# Autodesk Inventor assembly: robot
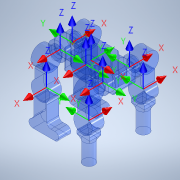
[picture p0: Inventor's stored thumbnail of the model, 180x180]
Saved by Autodesk Inventor 2020.2 (Build 242310000, 310)
## iProperties
Created: 2021-01-29
Part Number: robot
Document SubType Name: Assembly
Designer: DELL
Author: DELL
## Documents named in this file (6)
- D:\repo\FlexipodFast\mesh\v8.0\robot.iam
- D:\repo\FlexipodFast\mesh\v8.0\body.ipt
- D:\repo\FlexipodFast\mesh\v8.0\hip.ipt
- D:\repo\FlexipodFast\mesh\v8.0\thigh.ipt
- D:\repo\FlexipodFast\mesh\v8.0\shank_2.ipt
- D:\repo\FlexipodFast\mesh\v8.0\shank_front.ipt
## Components (13 placed, 5 different names)
1. body:1 — Flush:1, Flush:2, Flush:3, Mate:1, Mate:2, Mate:3, Mate:4, Angle:4, Angle:6, Angle:15, Angle:16, Angle:17, Angle:18, Mate:45, Mate:46, Mate:48, Mate:49, Angle:19, Angle:20, Angle:21, Angle:23, Angle:24, Angle:25, Angle:26, Angle:27, Angle:28, Angle:29, Angle:30, Angle:31
2. hip:1 — Mate:3, Mate:4, Angle:30, Flush:45, Mate:54
3. hip:2 — Mate:1, Mate:2, Angle:22, Angle:29, Mate:52, Mate:53
4. thigh:1 — Angle:17, Mate:44, Flush:43, Mate:52, Mate:53
5. thigh:2 — Angle:6, Mate:43, Flush:42, Angle:19, Angle:20, Flush:45, Mate:54
6. thigh:3 — Angle:16, Mate:42, Flush:41, Angle:23, Angle:24, Mate:55, Mate:56
7. thigh:4 — Angle:4, Angle:15, Angle:18, Mate:41, Flush:40, Angle:25, Angle:26, Mate:57, Flush:46
8. shank_2:3 — Mate:41, Flush:40, Angle:27
9. shank_2:4 — Mate:42, Flush:41, Angle:28
10. shank_front:1 — Mate:43, Flush:42, Angle:21
11. shank_front:2 — Mate:44, Flush:43, Angle:22
12. hip:3 — Mate:45, Mate:46, Mate:55, Angle:31, Mate:56
13. hip:4 — Mate:48, Mate:49, Mate:57, Flush:46
## Relationships (46: Angle 19, Mate 18, Flush 9)
- Flush:1: body:1
- Flush:2: body:1
- Flush:3: body:1
- Mate:1: body:1 ↔ hip:2
- Mate:2: body:1 ↔ hip:2
- Mate:3: body:1 ↔ hip:1
- Mate:4: body:1 ↔ hip:1
- Angle:4 (0 deg): body:1 ↔ thigh:4
- Angle:6 (0 deg): body:1 ↔ thigh:2
- Angle:15 (0 deg): body:1 ↔ thigh:4
- Angle:16 (0 deg): body:1 ↔ thigh:3
- Angle:17 (0 deg): body:1 ↔ thigh:1
- Angle:18 (0 deg): body:1 ↔ thigh:4
- Mate:41: thigh:4 ↔ shank_2:3
- Flush:40: thigh:4 ↔ shank_2:3
- Mate:42: thigh:3 ↔ shank_2:4
- Flush:41: thigh:3 ↔ shank_2:4
- Mate:43: thigh:2 ↔ shank_front:1
- Mate:44: thigh:1 ↔ shank_front:2
- Flush:42: thigh:2 ↔ shank_front:1
- Flush:43: thigh:1 ↔ shank_front:2
- Mate:45: body:1 ↔ hip:3
- Mate:46: body:1 ↔ hip:3
- Mate:48: body:1 ↔ hip:4
- Mate:49: body:1 ↔ hip:4
- Angle:19 (0 deg): body:1 ↔ thigh:2
- Angle:20 (0 deg): body:1 ↔ thigh:2
- Angle:21 (0 deg): body:1 ↔ shank_front:1
- Angle:22 (180 deg): hip:2 ↔ shank_front:2
- Angle:23 (0 deg): body:1 ↔ thigh:3
- Angle:24 (0 deg): body:1 ↔ thigh:3
- Angle:25 (0 deg): body:1 ↔ thigh:4
- Angle:26 (0 deg): body:1 ↔ thigh:4
- Angle:27 (0 deg): body:1 ↔ shank_2:3
- Angle:28 (0 deg): body:1 ↔ shank_2:4
- Angle:29 (0 deg): body:1 ↔ hip:2
- Mate:52: hip:2 ↔ thigh:1
- Mate:53: hip:2 ↔ thigh:1
- Angle:30 (0 deg): body:1 ↔ hip:1
- Flush:45: hip:1 ↔ thigh:2
- Mate:54: hip:1 ↔ thigh:2
- Mate:55: thigh:3 ↔ hip:3
- Angle:31 (0 deg): body:1 ↔ hip:3
- Mate:56: thigh:3 ↔ hip:3
- Mate:57: thigh:4 ↔ hip:4
- Flush:46: thigh:4 ↔ hip:4
